# Autodesk Inventor assembly: all_body
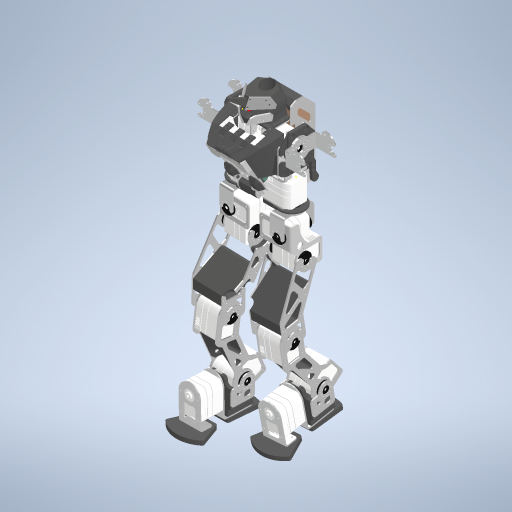
[picture p0: Inventor's stored thumbnail of the model, 512x512]
Saved by Autodesk Inventor 2024.1 (Build 281209000, 209)
## iProperties
Created: 2024-10-10
Part Number: all_body
Document SubType Name: Assembly
Designer: hibik
Author: hibik
## Documents named in this file (4)
- C:\Users\hibik\Documents\Robomech\HR\Eglantyne\hard\all_body.iam
- C:\Users\hibik\Documents\Robomech\HR\Eglantyne\hard\body.iam
- C:\Users\hibik\Documents\Robomech\HR\Eglantyne\hard\leg\leg_right.iam
- C:\Users\hibik\Documents\Robomech\HR\Eglantyne\hard\leg\leg_left.iam
## Components (3 placed, 3 different names)
1. body:1 [sub-assembly] — 挿入:1, 挿入:2
2. leg_right:1 [sub-assembly] — 挿入:1
3. leg_left:1 [sub-assembly] — 挿入:2
## Relationships (2: Insert 2)
- 挿入:1 [Insert]: body:1 ↔ leg_right:1
- 挿入:2 [Insert]: body:1 ↔ leg_left:1
